# Autodesk Inventor assembly: Shell draft 4
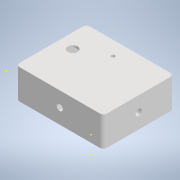
[picture p0: Inventor's stored thumbnail of the model, 180x180]
Saved by Autodesk Inventor 2022 (Build 260153000, 153)
## iProperties
Created: 2021-11-22
Part Number: Shell draft 4
Document SubType Name: Assembly
Designer: Elisabeth
Author: Elisabeth
## Documents named in this file (3)
- C:\Users\Elisabeth\Documents\SCHOOL\EE 491\Parts\Shell draft 4.iam
- C:\Users\Elisabeth\Documents\SCHOOL\EE 491\Parts\Shell 4 bottom.ipt
- C:\Users\Elisabeth\Documents\SCHOOL\EE 491\Parts\Shell 4 top.ipt
## Components (2 placed, 2 different names)
1. Shell 4 bottom:1 — Mate:1, Mate:2
2. Shell 4 top:1 — Mate:1, Mate:2
## Relationships (2: Mate 2)
- Mate:1: Shell 4 bottom:1 ↔ Shell 4 top:1
- Mate:2: Shell 4 bottom:1 ↔ Shell 4 top:1
